# Autodesk Inventor assembly: Y-Axis_new
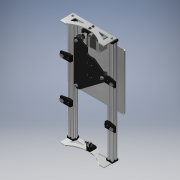
[picture p0: Inventor's stored thumbnail of the model, 180x180]
Saved by Autodesk Inventor 2020.3 (Build 243373000, 373)
## iProperties
Created: 2020-05-30
Part Number: Y-Axis_new
Document SubType Name: Assembly
Designer: rah75
Author: rah75
## Documents named in this file (19)
- C:\Users\rah75\Documents\GitHub\LETU-Maker\CAD\Autodesk Inventor\Base_3001-5999\Y-Axis\Assemblies\Y-Axis_Low_Profile_LM3049.iam
- C:\Users\rah75\Documents\GitHub\LETU-Maker\CAD\Autodesk Inventor\Base_3001-5999\Frame\Fabricated_Parts\Frame_Extrusion_20x20x400mm_LM3029.ipt
- C:\Users\rah75\Documents\GitHub\LETU-Maker\CAD\Autodesk Inventor\Base_3001-5999\Y-Axis\Fabricated_Parts\Y-Axis_Linear_Rod_1_4inx400mm_LM3038.ipt
- C:\Users\rah75\Documents\GitHub\LETU-Maker\CAD\Autodesk Inventor\Stock_Components_1001-2999\Motors\NEMA_17_LM1028.ipt
- C:\Users\rah75\Documents\GitHub\LETU-Maker\CAD\Autodesk Inventor\Stock_Components_1001-2999\Power_Transmission\GT2_pulley_LM1034.ipt
- C:\Users\rah75\Documents\GitHub\LETU-Maker\CAD\Autodesk Inventor\Base_3001-5999\Y-Axis\Printed_Parts\Y-Axis_Extrusion_Cap_LM3040.ipt
- C:\Users\rah75\Documents\GitHub\LETU-Maker\CAD\Autodesk Inventor\Base_3001-5999\Y-Axis\Printed_Parts\Y-Axis_Extursion_Mount_LM3041.ipt
- C:\Users\rah75\Documents\GitHub\LETU-Maker\CAD\Autodesk Inventor\Base_3001-5999\Y-Axis\Printed_Parts\Y-Axis_Motor_Mount_LM3042.ipt
- C:\Users\rah75\Documents\GitHub\LETU-Maker\CAD\Autodesk Inventor\Base_3001-5999\Y-Axis\Fabricated_Parts\Y-Axis_Cross_Bracket_LM3043.ipt
- C:\Users\rah75\Documents\GitHub\LETU-Maker\CAD\Autodesk Inventor\Base_3001-5999\Y-Axis\Printed_Parts\Y-Axis_Belt_Bearing_Mount_LM3045.ipt
- C:\Users\rah75\Documents\GitHub\LETU-Maker\CAD\Autodesk Inventor\Stock_Components_1001-2999\Power_Transmission\Bearings\625-ZZ_5x16mm_LM1030.ipt
- C:\Users\rah75\Documents\GitHub\LETU-Maker\CAD\Autodesk Inventor\Stock_Components_1001-2999\Electrical\limit_switch_LM1025.ipt
- C:\Users\rah75\Documents\GitHub\LETU-Maker\CAD\Autodesk Inventor\Base_3001-5999\Y-Carriage\Assemblies\Y-Carriage_Low_Profile_LM3050.iam
- C:\Users\rah75\Documents\GitHub\LETU-Maker\CAD\Autodesk Inventor\Stock_Components_1001-2999\Fasteners\Nuts\hex_nut_m5_LM1020.ipt
- C:\Users\rah75\Documents\GitHub\LETU-Maker\CAD\Autodesk Inventor\Stock_Components_1001-2999\Fasteners\Nuts\heat_insert_m5_LM1018.ipt
- C:\Users\rah75\Documents\GitHub\LETU-Maker\CAD\Autodesk Inventor\Stock_Components_1001-2999\Fasteners\Screws\BHHD_m5x25_LM1003.ipt
- C:\Users\rah75\Documents\GitHub\LETU-Maker\CAD\Autodesk Inventor\Stock_Components_1001-2999\Fasteners\Screws\BHHD_m5x10_LM1042.ipt
- C:\Users\rah75\Documents\GitHub\LETU-Maker\CAD\Autodesk Inventor\Stock_Components_1001-2999\Fasteners\Screws\BHHD_m5x15_LM1051.ipt
- C:\Users\rah75\Documents\GitHub\LETU-Maker\CAD\Autodesk Inventor\Stock_Components_1001-2999\Fasteners\Nuts\T_nut_m5_LM1021.ipt
## Components (51 placed, 18 different names)
1. Y-Axis_Cross_Bracket_LM3043:1 — Insert:3, Mate:19, Insert:12, Insert:30, Insert:31, Insert:32, Insert:33
2. Y-Axis_Cross_Bracket_LM3043:2 — Insert:1, Insert:2, Mate:17, Insert:18, Insert:26, Insert:27, Insert:28, Insert:29
3. Frame_Extrusion_20x20x400mm_LM3029:1 — Insert:2, Insert:3, Mate:2, Mate:4, Flush:1, Symmetry:1, Insert:8, Angle:3, Insert:9, Mate:15
4. Frame_Extrusion_20x20x400mm_LM3029:2 — Insert:1, Mate:1, Mate:3, Flush:2, Symmetry:1, Insert:7, Angle:2, Insert:10, Angle:4, Mate:14, Mate:16, Mate:21
5. Y-Axis_Linear_Rod_1_4inx400mm_LM3038:1 — Mate:2, Mate:5, Flush:1
6. Y-Axis_Linear_Rod_1_4inx400mm_LM3038:2 — Mate:1, Mate:3, Mate:4, Mate:5, Flush:2
7. NEMA_17_LM1028:1 — Insert:11, Insert:13
8. GT2_pulley_LM1034:1 — Insert:11
9. Y-Axis_Extrusion_Cap_LM3040:1 — Insert:7, Angle:2
10. Y-Axis_Extrusion_Cap_LM3040:2 — Insert:8, Angle:3
11. Y-Axis_Extrusion_Cap_LM3040:3 — Insert:9
12. Y-Axis_Extrusion_Cap_LM3040:4 — Insert:10, Angle:4
13. Y-Axis_Extursion_Mount_LM3041:1 — Flush:7, Flush:8, Flush:9, Mate:14, Flush:12, Flush:14, Mate:17, Insert:39, Insert:46
14. Y-Axis_Extursion_Mount_LM3041:2 — Flush:10, Flush:11, Flush:13, Insert:41, Insert:48
15. Y-Axis_Extursion_Mount_LM3041:3 — Flush:9, Flush:10, Flush:11, Mate:15, Flush:12, Insert:40, Insert:49
16. Y-Axis_Extursion_Mount_LM3041:4 — Flush:7, Flush:8, Mate:16, Flush:13, Flush:14, Insert:38, Insert:47
17. Y-Axis_Motor_Mount_LM3042:1 — Mate:19, Insert:12, Insert:13, Mate:22, Insert:20, Insert:21
18. Y-Axis_Belt_Bearing_Mount_LM3045:2 — Insert:18, Insert:19, Insert:22, Insert:23, Insert:24, Insert:25
19. 625-ZZ_5x16mm_LM1030:1 — Insert:19
20. limit_switch_LM1025:1
21. Y-Carriage_Low_Profile_LM3050:1 [sub-assembly] — Mate:20, Mate:21, Mate:22
22. hex_nut_m5_LM1020:1 — Insert:20
23. hex_nut_m5_LM1020:2 — Insert:21
24. heat_insert_m5_LM1018:1 — Insert:22
25. heat_insert_m5_LM1018:2 — Insert:23
26. BHHD_m5x25_LM1003:1 — Insert:24
27. hex_nut_m5_LM1020:3 — Insert:25
28. BHHD_m5x10_LM1042:1 — Insert:26
29. BHHD_m5x10_LM1042:2 — Insert:27
30. BHHD_m5x10_LM1042:3 — Insert:28
31. BHHD_m5x10_LM1042:4 — Insert:29
32. BHHD_m5x10_LM1042:5 — Insert:30
33. BHHD_m5x10_LM1042:6 — Insert:31
34. BHHD_m5x15_LM1051:1 — Insert:32
35. BHHD_m5x15_LM1051:2 — Insert:33
36. BHHD_m5x10_LM1042:7 — Insert:36, Insert:41
37. BHHD_m5x10_LM1042:8 — Insert:37, Insert:40
38. BHHD_m5x10_LM1042:9 — Insert:42, Insert:49
39. BHHD_m5x10_LM1042:10 — Insert:35, Insert:38
40. BHHD_m5x10_LM1042:11 — Insert:34, Insert:39
41. BHHD_m5x10_LM1042:12 — Insert:43, Insert:48
42. BHHD_m5x10_LM1042:13 — Insert:45, Insert:47
43. BHHD_m5x10_LM1042:14 — Insert:44, Insert:46
44. T_nut_m5_LM1021:1 — Insert:36, Mate:23
45. T_nut_m5_LM1021:2 — Insert:37, Mate:23
46. T_nut_m5_LM1021:3 — Insert:43, Mate:26
47. T_nut_m5_LM1021:4 — Insert:34, Mate:24
48. T_nut_m5_LM1021:5 — Insert:45, Mate:26
49. T_nut_m5_LM1021:6 — Insert:35, Mate:24
50. T_nut_m5_LM1021:7 — Insert:44, Mate:25
51. T_nut_m5_LM1021:8 — Insert:42, Mate:25
## Relationships (73: Insert 42, Mate 17, Flush 10, Angle 3, Symmetry 1)
- Insert:1 (2 mm): Y-Axis_Cross_Bracket_LM3043:2 ↔ Frame_Extrusion_20x20x400mm_LM3029:2
- Insert:2 (2 mm): Y-Axis_Cross_Bracket_LM3043:2 ↔ Frame_Extrusion_20x20x400mm_LM3029:1
- Insert:3 (2 mm): Y-Axis_Cross_Bracket_LM3043:1 ↔ Frame_Extrusion_20x20x400mm_LM3029:1
- Mate:1 (11.0395 mm): Frame_Extrusion_20x20x400mm_LM3029:2 ↔ Y-Axis_Linear_Rod_1_4inx400mm_LM3038:2
- Mate:2 (11.0395 mm): Frame_Extrusion_20x20x400mm_LM3029:1 ↔ Y-Axis_Linear_Rod_1_4inx400mm_LM3038:1
- Mate:3: Frame_Extrusion_20x20x400mm_LM3029:2 ↔ Y-Axis_Linear_Rod_1_4inx400mm_LM3038:2
- Mate:4: Frame_Extrusion_20x20x400mm_LM3029:1 ↔ Y-Axis_Linear_Rod_1_4inx400mm_LM3038:2
- Mate:5: Y-Axis_Linear_Rod_1_4inx400mm_LM3038:1 ↔ Y-Axis_Linear_Rod_1_4inx400mm_LM3038:2
- Flush:1: Frame_Extrusion_20x20x400mm_LM3029:1 ↔ Y-Axis_Linear_Rod_1_4inx400mm_LM3038:1
- Flush:2: Frame_Extrusion_20x20x400mm_LM3029:2 ↔ Y-Axis_Linear_Rod_1_4inx400mm_LM3038:2
- Symmetry:1: Frame_Extrusion_20x20x400mm_LM3029:1 ↔ Frame_Extrusion_20x20x400mm_LM3029:2
- Insert:7: Frame_Extrusion_20x20x400mm_LM3029:2 ↔ Y-Axis_Extrusion_Cap_LM3040:1
- Angle:2 (0 deg): Frame_Extrusion_20x20x400mm_LM3029:2 ↔ Y-Axis_Extrusion_Cap_LM3040:1
- Insert:8: Frame_Extrusion_20x20x400mm_LM3029:1 ↔ Y-Axis_Extrusion_Cap_LM3040:2
- Angle:3 (0 deg): Frame_Extrusion_20x20x400mm_LM3029:1 ↔ Y-Axis_Extrusion_Cap_LM3040:2
- Insert:9: Frame_Extrusion_20x20x400mm_LM3029:1 ↔ Y-Axis_Extrusion_Cap_LM3040:3
- Insert:10: Frame_Extrusion_20x20x400mm_LM3029:2 ↔ Y-Axis_Extrusion_Cap_LM3040:4
- Angle:4 (0 deg): Frame_Extrusion_20x20x400mm_LM3029:2 ↔ Y-Axis_Extrusion_Cap_LM3040:4
- Insert:11 (-16 mm): NEMA_17_LM1028:1 ↔ GT2_pulley_LM1034:1
- Flush:7: Y-Axis_Extursion_Mount_LM3041:1 ↔ Y-Axis_Extursion_Mount_LM3041:4
- Flush:8: Y-Axis_Extursion_Mount_LM3041:1 ↔ Y-Axis_Extursion_Mount_LM3041:4
- Flush:9: Y-Axis_Extursion_Mount_LM3041:1 ↔ Y-Axis_Extursion_Mount_LM3041:3
- Flush:10: Y-Axis_Extursion_Mount_LM3041:2 ↔ Y-Axis_Extursion_Mount_LM3041:3
- Flush:11: Y-Axis_Extursion_Mount_LM3041:2 ↔ Y-Axis_Extursion_Mount_LM3041:3
- Mate:14: Frame_Extrusion_20x20x400mm_LM3029:2 ↔ Y-Axis_Extursion_Mount_LM3041:1
- Mate:15: Frame_Extrusion_20x20x400mm_LM3029:1 ↔ Y-Axis_Extursion_Mount_LM3041:3
- Mate:16: Frame_Extrusion_20x20x400mm_LM3029:2 ↔ Y-Axis_Extursion_Mount_LM3041:4
- Flush:12: Y-Axis_Extursion_Mount_LM3041:1 ↔ Y-Axis_Extursion_Mount_LM3041:3
- Flush:13: Y-Axis_Extursion_Mount_LM3041:2 ↔ Y-Axis_Extursion_Mount_LM3041:4
- Flush:14 (150 mm): Y-Axis_Extursion_Mount_LM3041:1 ↔ Y-Axis_Extursion_Mount_LM3041:4
- Mate:17 (115 mm): Y-Axis_Cross_Bracket_LM3043:2 ↔ Y-Axis_Extursion_Mount_LM3041:1
- Mate:19: Y-Axis_Cross_Bracket_LM3043:1 ↔ Y-Axis_Motor_Mount_LM3042:1
- Insert:12: Y-Axis_Cross_Bracket_LM3043:1 ↔ Y-Axis_Motor_Mount_LM3042:1
- Insert:13: NEMA_17_LM1028:1 ↔ Y-Axis_Motor_Mount_LM3042:1
- Insert:18: Y-Axis_Cross_Bracket_LM3043:2 ↔ Y-Axis_Belt_Bearing_Mount_LM3045:2
- Insert:19 (1 mm): Y-Axis_Belt_Bearing_Mount_LM3045:2 ↔ 625-ZZ_5x16mm_LM1030:1
- Mate:20: Y-Carriage_Low_Profile_LM3050:1
- Mate:21 (3.5 mm): Frame_Extrusion_20x20x400mm_LM3029:2 ↔ Y-Carriage_Low_Profile_LM3050:1
- Mate:22: Y-Axis_Motor_Mount_LM3042:1 ↔ Y-Carriage_Low_Profile_LM3050:1
- Insert:20: Y-Axis_Motor_Mount_LM3042:1 ↔ hex_nut_m5_LM1020:1
- Insert:21: Y-Axis_Motor_Mount_LM3042:1 ↔ hex_nut_m5_LM1020:2
- Insert:22: Y-Axis_Belt_Bearing_Mount_LM3045:2 ↔ heat_insert_m5_LM1018:1
- Insert:23: Y-Axis_Belt_Bearing_Mount_LM3045:2 ↔ heat_insert_m5_LM1018:2
- Insert:24: Y-Axis_Belt_Bearing_Mount_LM3045:2 ↔ BHHD_m5x25_LM1003:1
- Insert:25: Y-Axis_Belt_Bearing_Mount_LM3045:2 ↔ hex_nut_m5_LM1020:3
- Insert:26: Y-Axis_Cross_Bracket_LM3043:2 ↔ BHHD_m5x10_LM1042:1
- Insert:27: Y-Axis_Cross_Bracket_LM3043:2 ↔ BHHD_m5x10_LM1042:2
- Insert:28: Y-Axis_Cross_Bracket_LM3043:2 ↔ BHHD_m5x10_LM1042:3
- Insert:29: Y-Axis_Cross_Bracket_LM3043:2 ↔ BHHD_m5x10_LM1042:4
- Insert:30: Y-Axis_Cross_Bracket_LM3043:1 ↔ BHHD_m5x10_LM1042:5
- Insert:31: Y-Axis_Cross_Bracket_LM3043:1 ↔ BHHD_m5x10_LM1042:6
- Insert:32: Y-Axis_Cross_Bracket_LM3043:1 ↔ BHHD_m5x15_LM1051:1
- Insert:33: Y-Axis_Cross_Bracket_LM3043:1 ↔ BHHD_m5x15_LM1051:2
- Insert:34 (6.25 mm): BHHD_m5x10_LM1042:11 ↔ T_nut_m5_LM1021:4
- Insert:35 (6.25 mm): BHHD_m5x10_LM1042:10 ↔ T_nut_m5_LM1021:6
- Insert:36 (6.25 mm): BHHD_m5x10_LM1042:7 ↔ T_nut_m5_LM1021:1
- Insert:37 (6.25 mm): BHHD_m5x10_LM1042:8 ↔ T_nut_m5_LM1021:2
- Insert:38: Y-Axis_Extursion_Mount_LM3041:4 ↔ BHHD_m5x10_LM1042:10
- Insert:39: Y-Axis_Extursion_Mount_LM3041:1 ↔ BHHD_m5x10_LM1042:11
- Mate:23: T_nut_m5_LM1021:1 ↔ T_nut_m5_LM1021:2
- Insert:40: Y-Axis_Extursion_Mount_LM3041:3 ↔ BHHD_m5x10_LM1042:8
- Insert:41: Y-Axis_Extursion_Mount_LM3041:2 ↔ BHHD_m5x10_LM1042:7
- Mate:24: T_nut_m5_LM1021:4 ↔ T_nut_m5_LM1021:6
- Insert:42 (6.5 mm): BHHD_m5x10_LM1042:9 ↔ T_nut_m5_LM1021:8
- Insert:43 (6.5 mm): BHHD_m5x10_LM1042:12 ↔ T_nut_m5_LM1021:3
- Insert:44 (6.5 mm): BHHD_m5x10_LM1042:14 ↔ T_nut_m5_LM1021:7
- Insert:45 (6.5 mm): BHHD_m5x10_LM1042:13 ↔ T_nut_m5_LM1021:5
- Mate:25: T_nut_m5_LM1021:7 ↔ T_nut_m5_LM1021:8
- Mate:26: T_nut_m5_LM1021:3 ↔ T_nut_m5_LM1021:5
- Insert:46: Y-Axis_Extursion_Mount_LM3041:1 ↔ BHHD_m5x10_LM1042:14
- Insert:47: Y-Axis_Extursion_Mount_LM3041:4 ↔ BHHD_m5x10_LM1042:13
- Insert:48: Y-Axis_Extursion_Mount_LM3041:2 ↔ BHHD_m5x10_LM1042:12
- Insert:49: Y-Axis_Extursion_Mount_LM3041:3 ↔ BHHD_m5x10_LM1042:9
